# Autodesk Inventor assembly: Assembly3
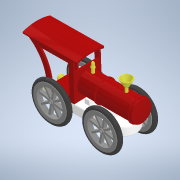
[picture p0: Inventor's stored thumbnail of the model, 180x180]
Saved by Autodesk Inventor 2021 (Build 250183000, 183)
## iProperties
Created: 2021-03-19
Part Number: Assembly3
Document SubType Name: Assembly
Designer: uriel
Author: uriel
## Documents named in this file (9)
- C:\Users\uriel\Documents\Escuela\LABORATORIO DISEÑO Y MANUFACTURA ASISTIDA POR COMPUTADORA\Practica 2\Assembly3.iam
- C:\Users\uriel\Documents\Escuela\LABORATORIO DISEÑO Y MANUFACTURA ASISTIDA POR COMPUTADORA\Practica 2\Assembly2.iam
- C:\Users\uriel\Documents\Escuela\LABORATORIO DISEÑO Y MANUFACTURA ASISTIDA POR COMPUTADORA\Practica 2\Imported Components\Base\Base.ipt
- C:\Users\uriel\Documents\Escuela\LABORATORIO DISEÑO Y MANUFACTURA ASISTIDA POR COMPUTADORA\Practica 2\Imported Components\Cabina\Cabina..ipt
- C:\Users\uriel\Documents\Escuela\LABORATORIO DISEÑO Y MANUFACTURA ASISTIDA POR COMPUTADORA\Practica 2\Imported Components\Cilindro\Cilindro.ipt
- C:\Users\uriel\Documents\Escuela\LABORATORIO DISEÑO Y MANUFACTURA ASISTIDA POR COMPUTADORA\Practica 2\Imported Components\Defensa\Defensa.ipt
- C:\Users\uriel\Documents\Escuela\LABORATORIO DISEÑO Y MANUFACTURA ASISTIDA POR COMPUTADORA\Practica 2\Imported Components\Eje\Eje.ipt
- C:\Users\uriel\Documents\Escuela\LABORATORIO DISEÑO Y MANUFACTURA ASISTIDA POR COMPUTADORA\Practica 2\Imported Components\Entrada\Entrada.ipt
- C:\Users\uriel\Documents\Escuela\LABORATORIO DISEÑO Y MANUFACTURA ASISTIDA POR COMPUTADORA\Practica 2\Imported Components\Salida\Salida.ipt
## Components (13 placed, 8 different names)
1. Assembly2:1 [sub-assembly] — Insert:6
2. Base:1 — Symmetry:1, Symmetry:2, Mate:5, Insert:1, Insert:2, Mate:7, Mate:8, Insert:3
3. Cabina.:1 — Mate:1, Angle:1, Symmetry:1, Symmetry:2, Mate:5, Angle:2
4. Cilindro:1 — Mate:1, Angle:1, Mate:2, Mate:3, Mate:4, Angle:2
5. Defensa:1 — Insert:3
6. Eje:1 — Insert:1, Insert:5, Insert:6
7. Entrada:1 — Mate:3, Mate:4
8. Salida:1 — Mate:2
9. Assembly2:2 [sub-assembly] — Insert:4
10. Assembly2:3 [sub-assembly] — Insert:7
11. Assembly2:4 [sub-assembly] — Insert:5
12. Defensa:2 — Mate:7, Mate:8
13. Eje:2 — Insert:2, Insert:4, Insert:7
## Relationships (18: Mate 7, Insert 7, Angle 2, Symmetry 2)
- Mate:1: Cabina.:1 ↔ Cilindro:1
- Angle:1 (0 deg): Cabina.:1 ↔ Cilindro:1
- Mate:2: Cilindro:1 ↔ Salida:1
- Mate:3: Cilindro:1 ↔ Entrada:1
- Mate:4: Cilindro:1 ↔ Entrada:1
- Symmetry:1: Base:1 ↔ Cabina.:1
- Symmetry:2: Base:1 ↔ Cabina.:1
- Mate:5: Base:1 ↔ Cabina.:1
- Insert:1 (-68.5 mm): Base:1 ↔ Eje:1
- Insert:2 (-68.5 mm): Base:1 ↔ Eje:2
- Mate:7: Base:1 ↔ Defensa:2
- Mate:8: Base:1 ↔ Defensa:2
- Insert:3: Base:1 ↔ Defensa:1
- Angle:2 (0 deg): Cabina.:1 ↔ Cilindro:1
- Insert:4 (-10 mm): Assembly2:2 ↔ Eje:2
- Insert:5 (-10 mm): Eje:1 ↔ Assembly2:4
- Insert:6 (-10 mm): Assembly2:1 ↔ Eje:1
- Insert:7 (-10 mm): Assembly2:3 ↔ Eje:2
